# Autodesk Inventor assembly: Assembly
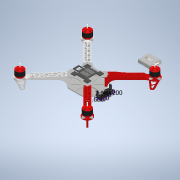
[picture p0: Inventor's stored thumbnail of the model, 180x180]
Saved by Autodesk Inventor 2020 (Build 240168000, 168)
## iProperties
Created: 2019-06-13
Part Number: Assembly
Document SubType Name: Assembly
Designer: amirt
Author: amirt
## Documents named in this file (8)
- C:\Users\amirt\Documents\Inventor\Drone\Assembly.iam
- C:\Users\amirt\Documents\Inventor\Drone\Frame.iam
- C:\Users\amirt\Documents\Inventor\Drone\Pixfalcon-Flight-Controller v1.ipt
- C:\Users\amirt\Documents\Inventor\Drone\Motor.iam
- C:\Users\amirt\Documents\Inventor\Drone\3DPrint\BatteryStopper.ipt
- C:\Users\amirt\Documents\Inventor\Drone\3DPrint\Part5.ipt
- C:\Users\amirt\Documents\Inventor\Drone\3DPrint\VibrationDampener.ipt
- C:\Users\amirt\Documents\Inventor\Drone\3DPrint\holder.ipt
## Components (11 placed, 7 different names)
1. Frame:1 [sub-assembly] — Mate:1, Mate:2, Mate:3, Mate:4, Mate:5, Flush:1, Flush:2, Flush:3, Mate:6, Flush:4, Mate:7, Flush:6, Flush:7
2. Pixfalcon-Flight-Controller v1:1 — Mate:1
3. BatteryStopper:1 — Mate:5, Flush:1
4. Part5:1 — Flush:2
5. VibrationDampener:1 — Flush:4, Mate:7, Flush:5
6. VibrationDampener:2 — Flush:3, Mate:6, Flush:5, Flush:6
7. holder:1 — Flush:7
8. Motor:1 [sub-assembly] — Mate:3, Mate:4
9. Motor:2 [sub-assembly]
10. Motor:3 [sub-assembly]
11. Motor:4 [sub-assembly]
## Component patterns: (4 elements, first: Motor:1)
## Relationships (14: Mate 7, Flush 7)
- Mate:1: Frame:1 ↔ Pixfalcon-Flight-Controller v1:1
- Mate:2: Frame:1
- Mate:3: Frame:1 ↔ Motor:1
- Mate:4: Frame:1 ↔ Motor:1
- Mate:5: Frame:1 ↔ BatteryStopper:1
- Flush:1 (-1.5875 mm): Frame:1 ↔ BatteryStopper:1
- Flush:2: Frame:1 ↔ Part5:1
- Flush:3: Frame:1 ↔ VibrationDampener:2
- Mate:6: Frame:1 ↔ VibrationDampener:2
- Flush:4: Frame:1 ↔ VibrationDampener:1
- Mate:7: Frame:1 ↔ VibrationDampener:1
- Flush:5: VibrationDampener:1 ↔ VibrationDampener:2
- Flush:6 (1.524 mm): Frame:1 ↔ VibrationDampener:2
- Flush:7: Frame:1 ↔ holder:1
